# Autodesk Inventor assembly: left_foot_link_MIR
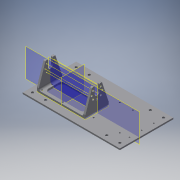
[picture p0: Inventor's stored thumbnail of the model, 180x180]
Saved by Autodesk Inventor 2018 (Build 220112000, 112)
## iProperties
Created: 2018-11-30
Part Number: left_foot_link_MIR
Document SubType Name: Assembly
Designer: bitbots
Author: bitbots
## Documents named in this file (3)
- C:\Users\jaspe\bitbots_hardware\wolfgang\assembly\legs\left_foot_link_MIR.iam
- C:\Users\jaspe\bitbots_hardware\wolfgang\assembly\legs\ankle_MIR_MIR_MIR.ipt
- C:\Users\jaspe\bitbots_hardware\wolfgang\assembly\legs\foot_MIR_MIR_MIR.ipt
## Components (2 placed, 2 different names)
1. ankle_MIR_MIR_MIR:1 — Flush:1, Mate:3, Mate:2, Mate:1, Mate:5, Mate:4, Mate:8, Mate:9
2. foot_MIR_MIR_MIR:1 — Mate:3, Mate:2, Mate:1, Angle:1
## Relationships (9: Mate 8, Angle 1)
- Flush:1 [Mate]: ankle_MIR_MIR_MIR:1
- Mate:3: ankle_MIR_MIR_MIR:1 ↔ foot_MIR_MIR_MIR:1
- Mate:2: ankle_MIR_MIR_MIR:1 ↔ foot_MIR_MIR_MIR:1
- Mate:1: ankle_MIR_MIR_MIR:1 ↔ foot_MIR_MIR_MIR:1
- Mate:5: ankle_MIR_MIR_MIR:1
- Mate:4: ankle_MIR_MIR_MIR:1
- Mate:8 (92 mm): ankle_MIR_MIR_MIR:1
- Mate:9 (7.139 mm): ankle_MIR_MIR_MIR:1
- Angle:1 (0 deg): foot_MIR_MIR_MIR:1
